# Autodesk Inventor assembly: Pit Station
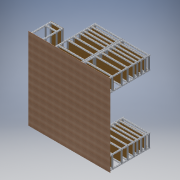
[picture p0: Inventor's stored thumbnail of the model, 180x180]
Saved by Autodesk Inventor 2019.4 (Build 234330000, 330)
## iProperties
Created: 2020-02-27
Part Number: Pit Station
Document SubType Name: Assembly
Designer: admin
Author: admin
## Documents named in this file (5)
- C:\Users\admin\Desktop\FRC 2020 Engineering\GitHub\7738-2020\Pit Station Designs\Pit Station.iam
- C:\Users\admin\Desktop\FRC 2020 Engineering\GitHub\7738-2020\Pit Station Designs\Pit Station floor.ipt
- C:\Users\admin\Desktop\FRC 2020 Engineering\GitHub\7738-2020\Pit Station Designs\Table\Table Assembly.iam
- C:\Users\admin\Desktop\FRC 2020 Engineering\GitHub\7738-2020\Pit Station Designs\battery rack\Battery Rack Assembly.iam
- C:\Users\admin\Desktop\FRC 2020 Engineering\GitHub\7738-2020\Pit Station Designs\Storage racks\Storage Rack Assembly.iam
## Components (7 placed, 4 different names)
1. Pit Station floor:1 — Mate:1, Mate:2, Mate:5, Mate:6, Mate:7, Mate:8
2. Table Assembly:1 [sub-assembly] — Mate:1, Mate:3, Flush:1
3. Table Assembly:2 [sub-assembly] — Mate:2, Mate:3, Flush:1
4. Storage Rack Assembly:1 [sub-assembly] — Mate:6
5. Storage Rack Assembly:2 [sub-assembly] — Mate:7
6. Storage Rack Assembly:3 [sub-assembly] — Mate:5
7. Battery Rack Assembly:2 [sub-assembly] — Mate:8
## Relationships (8: Mate 7, Flush 1)
- Mate:1: Pit Station floor:1 ↔ Table Assembly:1
- Mate:2: Pit Station floor:1 ↔ Table Assembly:2
- Mate:3: Table Assembly:1 ↔ Table Assembly:2
- Flush:1: Table Assembly:1 ↔ Table Assembly:2
- Mate:5: Pit Station floor:1 ↔ Storage Rack Assembly:3
- Mate:6: Pit Station floor:1 ↔ Storage Rack Assembly:1
- Mate:7: Pit Station floor:1 ↔ Storage Rack Assembly:2
- Mate:8: Pit Station floor:1 ↔ Battery Rack Assembly:2
